# Autodesk Inventor assembly: 하단 조립품
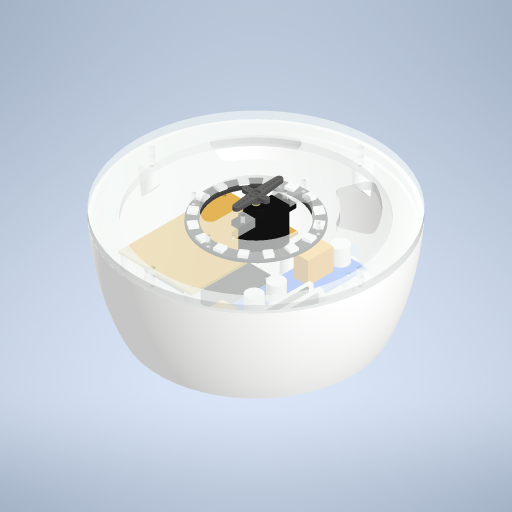
[picture p0: Inventor's stored thumbnail of the model, 512x512]
Saved by Autodesk Inventor 2023 (Build 270158000, 158)
## iProperties
Created: 2022-08-10
Part Number: 하단 조립품
Document SubType Name: Assembly
Designer: fly01
Author: fly01
## Documents named in this file (8)
- C:\Users\user\Desktop\PAI\PAI설계\조림품\하단 조립품.iam
- C:\Users\user\Desktop\PAI\PAI설계\출력품\body_bottom.ipt
- C:\Users\user\Desktop\PAI\PAI설계\조림품\하단 아크릴 조립품.iam
- C:\Users\user\Desktop\PAI\PAI설계\범용 부품\육각렌치볼트 m3 15mm.ipt
- C:\Users\user\Desktop\PAI\PAI설계\범용 부품\더블 릴레이 모듈.ipt
- C:\Users\user\Desktop\PAI\PAI설계\범용 부품\만능기판 소형.ipt
- C:\Users\user\Desktop\PAI\PAI설계\범용 부품\블루투스 모듈.ipt
- C:\Users\user\Desktop\PAI\PAI설계\범용 부품\스텝다운 컨버터.ipt
## Components (12 placed, 7 different names)
1. body_bottom:1 — 삽입:1, 삽입:2, 삽입:6, 삽입:7, 메이트:1, 메이트:2, 메이트:3, 메이트:4, 삽입:12, 삽입:13, 삽입:14, 삽입:15, 삽입:16, 삽입:17
2. 하단 아크릴 조립품:1 [sub-assembly] — 삽입:1, 삽입:2, 삽입:3
3. 더블 릴레이 모듈:1 — 삽입:12, 삽입:13
4. 만능기판 소형:1 — 삽입:6, 삽입:7
5. 블루투스 모듈:1 — 메이트:1, 메이트:2
6. 블루투스 모듈:3 — 메이트:3, 메이트:4
7. 스텝다운 컨버터:1 — 삽입:14, 삽입:15
8. 스텝다운 컨버터:2 — 삽입:16, 삽입:17
9. 육각렌치볼트 m3 15mm:1 — 삽입:3
10. 육각렌치볼트 m3 15mm:2
11. 육각렌치볼트 m3 15mm:3
12. 육각렌치볼트 m3 15mm:4
## Component patterns: (4 elements, first: 육각렌치볼트 m3 15mm:1)
## Relationships (15: Insert 11, Mate 4)
- 삽입:1 [Insert] (-5 mm): body_bottom:1 ↔ 하단 아크릴 조립품:1
- 삽입:2 [Insert]: body_bottom:1 ↔ 하단 아크릴 조립품:1
- 삽입:3 [Insert]: 하단 아크릴 조립품:1 ↔ 육각렌치볼트 m3 15mm:1
- 삽입:6 [Insert]: body_bottom:1 ↔ 만능기판 소형:1
- 삽입:7 [Insert]: body_bottom:1 ↔ 만능기판 소형:1
- 메이트:1 [Mate]: body_bottom:1 ↔ 블루투스 모듈:1
- 메이트:2 [Mate]: body_bottom:1 ↔ 블루투스 모듈:1
- 메이트:3 [Mate]: body_bottom:1 ↔ 블루투스 모듈:3
- 메이트:4 [Mate]: body_bottom:1 ↔ 블루투스 모듈:3
- 삽입:12 [Insert]: body_bottom:1 ↔ 더블 릴레이 모듈:1
- 삽입:13 [Insert]: body_bottom:1 ↔ 더블 릴레이 모듈:1
- 삽입:14 [Insert]: body_bottom:1 ↔ 스텝다운 컨버터:1
- 삽입:15 [Insert]: body_bottom:1 ↔ 스텝다운 컨버터:1
- 삽입:16 [Insert]: body_bottom:1 ↔ 스텝다운 컨버터:2
- 삽입:17 [Insert]: body_bottom:1 ↔ 스텝다운 컨버터:2
